# Autodesk Inventor assembly: Functioning swerve drive (motor)
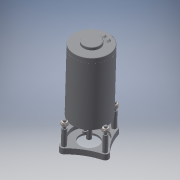
[picture p0: Inventor's stored thumbnail of the model, 180x180]
Saved by Autodesk Inventor 2019 (Build 230136000, 136)
## iProperties
Created: 2019-01-14
Part Number: Functioning swerve drive (motor)
Document SubType Name: Assembly
Designer: josh
Mass: 403.105 g
Surface Area: 533.836 cm^2
Volume: 400.712 cm^3
Density: 1.00597 g/cm^3
Author: josh
## Documents named in this file (7)
- D:\Synthesis Robots\Epsilon\Functioning swerve drive sub-assemblies\Functioning swerve drive (motor).iam
- D:\Synthesis Robots\Epsilon\Swerve drive parts\CIM Motor SW.ipt
- D:\Synthesis Robots\Epsilon\Swerve drive parts\10-32x0625_shcs_HX-SHCS 0.19-32x1.375x1-C.ipt
- D:\Synthesis Robots\Epsilon\Swerve drive parts\1100x215 alum spacer 83062 K-S.ipt
- D:\Synthesis Robots\Epsilon\Epsilon elavator lift\Functioning elevator parts\10-32 Nylock Nut.ipt
- D:\Synthesis Robots\Epsilon\Swerve drive parts\10-32x1750_shcs_HX-SHCS 0.19-32x1.375x1-C.ipt
- D:\Synthesis Robots\Epsilon\Swerve drive parts\Bearing Plate.ipt
## Components (16 placed, 6 different names)
1. CIM Motor SW:1
2. 10-32x1750_shcs_HX-SHCS 0.19-32x1.375x1-C:4
3. Bearing Plate:1
4. 10-32x1750_shcs_HX-SHCS 0.19-32x1.375x1-C:1
5. 1100x215 alum spacer 83062 K-S:1
6. 10-32 Nylock Nut:2
7. 1100x215 alum spacer 83062 K-S:2
8. 1100x215 alum spacer 83062 K-S:3
9. 10-32 Nylock Nut:4
10. 10-32x1750_shcs_HX-SHCS 0.19-32x1.375x1-C:3
11. 10-32x1750_shcs_HX-SHCS 0.19-32x1.375x1-C:2
12. 1100x215 alum spacer 83062 K-S:4
13. 10-32 Nylock Nut:3
14. 10-32 Nylock Nut:1
15. 10-32x0625_shcs_HX-SHCS 0.19-32x1.375x1-C:1
16. 10-32x0625_shcs_HX-SHCS 0.19-32x1.375x1-C:2
## Relationships (18: Mate 18)
- [Mate]: CIM Motor SW:1 ↔ 10-32x0625_shcs_HX-SHCS 0.19-32x1.375x1-C:2
- [Mate]: CIM Motor SW:1 ↔ 10-32x0625_shcs_HX-SHCS 0.19-32x1.375x1-C:1
- [Mate]: 1100x215 alum spacer 83062 K-S:3 ↔ 10-32x1750_shcs_HX-SHCS 0.19-32x1.375x1-C:3
- [Mate]: Bearing Plate:1 ↔ 10-32x1750_shcs_HX-SHCS 0.19-32x1.375x1-C:3
- [Mate]: Bearing Plate:1 ↔ 10-32x1750_shcs_HX-SHCS 0.19-32x1.375x1-C:3
- [Mate]: 10-32x1750_shcs_HX-SHCS 0.19-32x1.375x1-C:4 ↔ 1100x215 alum spacer 83062 K-S:2
- [Mate]: 10-32x1750_shcs_HX-SHCS 0.19-32x1.375x1-C:4 ↔ Bearing Plate:1
- [Mate]: Bearing Plate:1 ↔ 1100x215 alum spacer 83062 K-S:2
- [Mate]: 10-32x1750_shcs_HX-SHCS 0.19-32x1.375x1-C:4 ↔ Bearing Plate:1
- [Mate]: Bearing Plate:1 ↔ 1100x215 alum spacer 83062 K-S:3
- [Mate]: Bearing Plate:1 ↔ 10-32x1750_shcs_HX-SHCS 0.19-32x1.375x1-C:1
- [Mate]: Bearing Plate:1 ↔ 10-32x1750_shcs_HX-SHCS 0.19-32x1.375x1-C:1
- [Mate]: 10-32x1750_shcs_HX-SHCS 0.19-32x1.375x1-C:1 ↔ 1100x215 alum spacer 83062 K-S:1
- [Mate]: Bearing Plate:1 ↔ 1100x215 alum spacer 83062 K-S:1
- [Mate]: Bearing Plate:1 ↔ 10-32x1750_shcs_HX-SHCS 0.19-32x1.375x1-C:2
- [Mate]: Bearing Plate:1 ↔ 10-32x1750_shcs_HX-SHCS 0.19-32x1.375x1-C:2
- [Mate]: 10-32x1750_shcs_HX-SHCS 0.19-32x1.375x1-C:2 ↔ 1100x215 alum spacer 83062 K-S:4
- [Mate]: Bearing Plate:1 ↔ 1100x215 alum spacer 83062 K-S:4
## Named parameters: d14_d376_d243 = 0 mm, d15_d379_d246 = 0 mm, d373_d240 = 0 mm, d374_d241 = 0 mm, d174_d222 = 0 mm, d175_d223 = 0 mm, d176_d224 = 0 mm, d177_d225 = 0 mm, d178_d226 = 0 mm, d180_d227 = 0 mm, d181_d228 = 0 mm, d183_d230 = 0 mm, d365_d232 = 0 mm, d368_d235 = 0 mm, d369_d236 = 0 mm, d370_d237 = 0 mm, d371_d238 = 0 mm, d372_d239 = 0 mm
